# Autodesk Inventor assembly: ammoTinenclosure.ipt
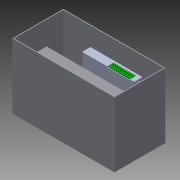
[picture p0: Inventor's stored thumbnail of the model, 180x180]
Saved by Autodesk Inventor 2013 (Build 170138000, 138)
## iProperties
Created: 2013-03-14
Part Number: ammoTinenclosure.ipt
Document SubType Name: Assembly
Designer: james.eddlestone
Author: james.eddlestone
## Documents named in this file (4)
- C:\Users\james.eddlestone\Documents\GitHub\Crown-Fire\CAD\Electronics\Enclosure\ammoTinenclosure.ipt.iam
- C:\Users\james.eddlestone\Documents\GitHub\Crown-Fire\CAD\Electronics\Enclosure\ammoTin.ipt
- C:\Users\james.eddlestone\Documents\GitHub\Crown-Fire\CAD\Electronics\Controller\Geckdrive G540\Geckdrive G540.iam
- C:\Users\james.eddlestone\Documents\GitHub\Crown-Fire\CAD\Electronics\powerSupply.ipt
## Components (3 placed, 3 different names)
1. ammoTin:1 — Mate:1, Flush:1, Mate:2, Mate:3, Flush:2, Flush:3
2. Geckdrive G540:1 [sub-assembly] — Mate:3, Flush:2, Flush:3
3. powerSupply:1 — Mate:1, Flush:1, Mate:2
## Relationships (6: Mate 3, Flush 3)
- Mate:1: ammoTin:1 ↔ powerSupply:1
- Flush:1 (25.4 mm): ammoTin:1 ↔ powerSupply:1
- Mate:2 (25.4 mm): ammoTin:1 ↔ powerSupply:1
- Mate:3: ammoTin:1 ↔ Geckdrive G540:1
- Flush:2 (-50.8 mm): ammoTin:1 ↔ Geckdrive G540:1
- Flush:3 (50.8 mm): ammoTin:1 ↔ Geckdrive G540:1
